# Autodesk Inventor assembly: Beta Motor Assembly
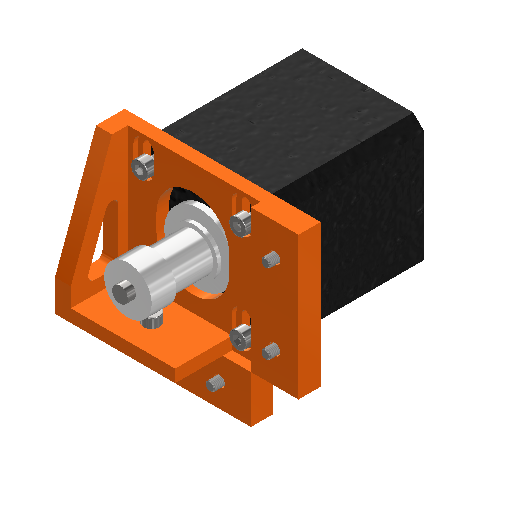
[picture p0: Inventor's stored thumbnail of the model, 512x512]
Saved by Autodesk Inventor 2023.2 (Build 272271000, 271)
## iProperties
Created: 2023-02-03
Part Number: Beta Motor Assembly
Document SubType Name: Assembly
Designer: remop
Author: remop
## Documents named in this file (5)
- C:\Users\remop\OneDrive\Documents\Inventor\3D Printers\LuEVO\Mk5_FullKinematic\Beta Motor Assembly.iam
- C:\Users\remop\OneDrive\Documents\Inventor\3D Printers\LuEVO\Mk5_FullKinematic\Beta Motor Mount.ipt
- C:\Users\remop\OneDrive\Documents\Inventor\3D Printers\LuEVO\Mk5_FullKinematic\XY Axis Motor (Stepper).ipt
- C:\Users\remop\OneDrive\Documents\Inventor\3D Printers\LuEVO\Mk5_FullKinematic\Belt Pulley.ipt
- C:\Users\remop\OneDrive\Documents\Inventor\Content Center Files\R2023\en-US\AS 1420\AS 1420 - 1973 - M3 x 6.ipt
## Components (12 placed, 4 different names)
1. Beta Motor Mount:1 — Rigid:3, Insert:4, Insert:5, Insert:6, Insert:7, Insert:8, Insert:11, Insert:13, Insert:15, Insert:16
2. XY Axis Motor (Stepper):1 — Rigid:2, Rigid:3
3. Belt Pulley:1 — Rigid:2
4. AS 1420 - Metric M3 x 6:4 — Insert:4
5. AS 1420 - Metric M3 x 6:5 — Insert:5
6. AS 1420 - Metric M3 x 6:6 — Insert:6
7. AS 1420 - Metric M3 x 6:7 — Insert:7
8. AS 1420 - Metric M3 x 6:8 — Insert:8
9. AS 1420 - Metric M3 x 6:11 — Insert:11
10. AS 1420 - Metric M3 x 6:13 — Insert:13
11. AS 1420 - Metric M3 x 6:15 — Insert:15
12. AS 1420 - Metric M3 x 6:16 — Insert:16
## Relationships (11: Insert 9, WeldJoint 2)
- Rigid:2 [WeldJoint] (-0.5 mm): XY Axis Motor (Stepper):1 ↔ Belt Pulley:1
- Rigid:3 [WeldJoint]: Beta Motor Mount:1 ↔ XY Axis Motor (Stepper):1
- Insert:4: Beta Motor Mount:1 ↔ AS 1420 - Metric M3 x 6:4
- Insert:5: Beta Motor Mount:1 ↔ AS 1420 - Metric M3 x 6:5
- Insert:6: Beta Motor Mount:1 ↔ AS 1420 - Metric M3 x 6:6
- Insert:7: Beta Motor Mount:1 ↔ AS 1420 - Metric M3 x 6:7
- Insert:8: Beta Motor Mount:1 ↔ AS 1420 - Metric M3 x 6:8
- Insert:11: Beta Motor Mount:1 ↔ AS 1420 - Metric M3 x 6:11
- Insert:13: Beta Motor Mount:1 ↔ AS 1420 - Metric M3 x 6:13
- Insert:15: Beta Motor Mount:1 ↔ AS 1420 - Metric M3 x 6:15
- Insert:16: Beta Motor Mount:1 ↔ AS 1420 - Metric M3 x 6:16
